# Autodesk Inventor assembly: Pista Orizzontale
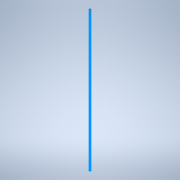
[picture p0: Inventor's stored thumbnail of the model, 180x180]
Saved by Autodesk Inventor 2022 (Build 260153000, 153)
## iProperties
Created: 2021-12-30
Part Number: Pista Orizzontale
Document SubType Name: Assembly
Designer: matte
Author: matte
## Documents named in this file (4)
- C:\Users\matte\Documents\GitHub\MDM-CyberOrto-CAD\Pezzi singoli\Pista Orizzontale.iam
- C:\Users\matte\Documents\GitHub\MDM-CyberOrto-CAD\Pezzi singoli\Supporto lineare\Binario.ipt
- C:\Users\matte\Documents\GitHub\MDM-CyberOrto-CAD\Pezzi singoli\Supporto lineare\Clamp.ipt
- C:\Users\matte\Documents\GitHub\MDM-CyberOrto-CAD\Pezzi singoli\Supporto lineare\Shaft.ipt
## Components (5 placed, 5 different names)
1. Binario:1
2. Clamp DX
3. Shaft DX
4. Clamp SX
5. Shaft SX
## Relationships (12: Flush 7, Mate 2, Tangent 2, Symmetry 1)
- [Flush]: Binario:1 ↔ Clamp DX
- [Mate]: Binario:1 ↔ Clamp DX
- [Mate]: Binario:1 ↔ Clamp DX
- [Flush]: Clamp DX ↔ Shaft DX
- [Flush]: Clamp DX ↔ Shaft DX
- [Tangent]: Clamp DX ↔ Shaft DX
- [Flush]: Clamp SX ↔ Shaft SX
- [Flush]: Clamp SX ↔ Shaft SX
- [Tangent]: Clamp SX ↔ Shaft SX
- [Symmetry]: Clamp DX ↔ Clamp SX
- [Flush]: Shaft DX ↔ Shaft SX
- [Flush]: Shaft DX ↔ Shaft SX
## Named parameters: d0_d8 = 0 mm, d1_d9 = 0 mm, d2_d10 = 0 mm, d11_d8 = 0 mm, d12_d9 = 0 mm, d13_d10 = 0 mm
